# Autodesk Inventor assembly: locomotion assembly-01
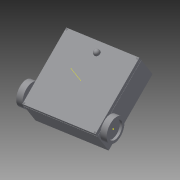
[picture p0: Inventor's stored thumbnail of the model, 180x180]
Saved by Autodesk Inventor 2015 (Build 190159000, 159)
## iProperties
Created: 2014-10-11
Part Number: locomotion assembly-01
Document SubType Name: Assembly
Designer: ericd_000
Author: ericd_000
## Documents named in this file (12)
- C:\Users\ericd_000\Dropbox\GitHub\initial_cad\eric_cad\locomotion assembly\locomotion assembly-01.iam
- C:\Users\ericd_000\Dropbox\GitHub\initial_cad\eric_cad\locomotion box.ipt
- C:\Users\ericd_000\Dropbox\GitHub\initial_cad\eric_cad\male bayonet connector 10.ipt
- C:\Users\ericd_000\Dropbox\GitHub\initial_cad\eric_cad\Imported Components\217-2000\217-2000.ipt
- C:\Users\ericd_000\Dropbox\GitHub\initial_cad\eric_cad\stark24v10ahbattery.ipt
- C:\Users\ericd_000\Dropbox\GitHub\initial_cad\eric_cad\udoo.ipt
- C:\Users\ericd_000\Dropbox\GitHub\initial_cad\eric_cad\Imported Components\M4 10mm length\M4 10mm length.ipt
- C:\Users\ericd_000\Dropbox\GitHub\initial_cad\eric_cad\100mm wheel.ipt
- C:\Users\ericd_000\Dropbox\GitHub\initial_cad\eric_cad\power board.ipt
- C:\Users\ericd_000\Dropbox\GitHub\initial_cad\eric_cad\locomotion top.ipt
- C:\Users\ericd_000\Dropbox\GitHub\initial_cad\eric_cad\Imported Components\M4 18mm\M4 18mm.ipt
- C:\Users\ericd_000\Dropbox\GitHub\initial_cad\eric_cad\locomotion assembly.iam
## Components (18 placed, 10 different names)
1. locomotion box:1 — Mate:1, Cylindrical:1, Cylindrical:2, Cylindrical:4, Cylindrical:6, Mate:5, Mate:6, Mate:7, Cylindrical:8, Cylindrical:9, Mate:8, Mate:9, Mate:10, Mate:12, Mate:13, Cylindrical:18, Cylindrical:19, Mate:16, Mate:21, Mate:22
2. male bayonet connector 10:1 — Mate:1, Cylindrical:1, Cylindrical:2
3. 217-2000:1 — Cylindrical:10, Cylindrical:11, Mate:8, Cylindrical:13, Mate:11
4. 217-2000:2 — Cylindrical:5, Cylindrical:7, Mate:5, Cylindrical:12, Flush:1
5. stark24v10ahbattery:1 — Mate:15, Mate:21, Mate:22, Flush:2
6. udoo:1 — Mate:12, Mate:14, Mate:15, Flush:2
7. M4 10mm length:1 — Cylindrical:6, Cylindrical:7, Mate:7
8. M4 10mm length:2 — Cylindrical:4, Cylindrical:5, Mate:6
9. M4 10mm length:3 — Cylindrical:8, Cylindrical:11, Mate:10
10. M4 10mm length:4 — Cylindrical:9, Cylindrical:10, Mate:9
11. 100mm wheel:1 — Cylindrical:12, Flush:1
12. 100mm wheel:2 — Cylindrical:13, Mate:11
13. power board:1 — Mate:13, Mate:14
14. locomotion top:1 — Cylindrical:14, Cylindrical:15, Cylindrical:16, Cylindrical:17, Mate:16, Mate:17, Mate:18, Mate:19, Mate:20
15. M4 18mm:1 — Cylindrical:17, Cylindrical:19, Mate:19
16. M4 18mm:2 — Cylindrical:14, Mate:17
17. M4 18mm:3 — Cylindrical:16, Mate:20
18. M4 18mm:4 — Cylindrical:15, Cylindrical:18, Mate:18
## Relationships (39: Mate 19, CylindricalJoint 18, Flush 2)
- Mate:1: locomotion box:1 ↔ male bayonet connector 10:1
- Cylindrical:1: locomotion box:1 ↔ male bayonet connector 10:1
- Cylindrical:2: locomotion box:1 ↔ male bayonet connector 10:1
- Cylindrical:4: locomotion box:1 ↔ M4 10mm length:2
- Cylindrical:5: 217-2000:2 ↔ M4 10mm length:2
- Cylindrical:6: locomotion box:1 ↔ M4 10mm length:1
- Cylindrical:7: 217-2000:2 ↔ M4 10mm length:1
- Mate:5 (0.1 mm): locomotion box:1 ↔ 217-2000:2
- Mate:6: locomotion box:1 ↔ M4 10mm length:2
- Mate:7: locomotion box:1 ↔ M4 10mm length:1
- Cylindrical:8: locomotion box:1 ↔ M4 10mm length:3
- Cylindrical:9: locomotion box:1 ↔ M4 10mm length:4
- Cylindrical:10: 217-2000:1 ↔ M4 10mm length:4
- Cylindrical:11: 217-2000:1 ↔ M4 10mm length:3
- Mate:8 (0.1 mm): locomotion box:1 ↔ 217-2000:1
- Mate:9: locomotion box:1 ↔ M4 10mm length:4
- Mate:10: locomotion box:1 ↔ M4 10mm length:3
- Cylindrical:12: 217-2000:2 ↔ 100mm wheel:1
- Flush:1 (0.1 mm): 217-2000:2 ↔ 100mm wheel:1
- Cylindrical:13: 217-2000:1 ↔ 100mm wheel:2
- Mate:11 (0.1 mm): 217-2000:1 ↔ 100mm wheel:2
- Mate:12 (1 mm): locomotion box:1 ↔ udoo:1
- Mate:13 (1 mm): locomotion box:1 ↔ power board:1
- Mate:14 (4 mm): udoo:1 ↔ power board:1
- Mate:15 (3 mm): stark24v10ahbattery:1 ↔ udoo:1
- Cylindrical:14: locomotion top:1 ↔ M4 18mm:2
- Cylindrical:15: locomotion top:1 ↔ M4 18mm:4
- Cylindrical:16: locomotion top:1 ↔ M4 18mm:3
- Cylindrical:17: locomotion top:1 ↔ M4 18mm:1
- Cylindrical:18: locomotion box:1 ↔ M4 18mm:4
- Cylindrical:19: locomotion box:1 ↔ M4 18mm:1
- Mate:16: locomotion box:1 ↔ locomotion top:1
- Mate:17: locomotion top:1 ↔ M4 18mm:2
- Mate:18: locomotion top:1 ↔ M4 18mm:4
- Mate:19: locomotion top:1 ↔ M4 18mm:1
- Mate:20: locomotion top:1 ↔ M4 18mm:3
- Mate:21 (60 mm): locomotion box:1 ↔ stark24v10ahbattery:1
- Mate:22 (20 mm): locomotion box:1 ↔ stark24v10ahbattery:1
- Flush:2 (37 mm): stark24v10ahbattery:1 ↔ udoo:1
